# Autodesk Inventor assembly: コックピット_1
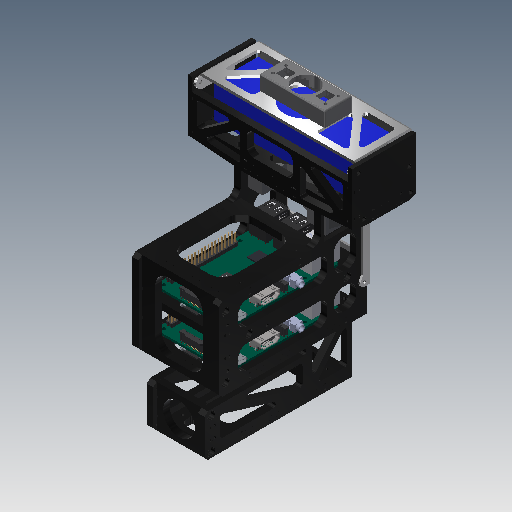
[picture p0: Inventor's stored thumbnail of the model, 512x512]
Saved by Autodesk Inventor 2017.3 (Build 213256000, 256)
## iProperties
Created: 2016-05-08
Part Number: コックピット_1
Document SubType Name: Assembly
Designer: hiroaki
Mass: 626.642 g
Surface Area: 2154.4 cm^2
Volume: 306.453 cm^3
Density: 2.04482 g/cm^3
Author: hiroaki
## Documents named in this file (19)
- C:\Users\haya\Desktop\GankenKun0_5\上半身\コックピット\コックピット_2\コックピット_2.iam
- C:\Users\haya\Desktop\GankenKun0_5\インポートされたコンポーネント\raspberrypi_b_+_(assembly)\raspberrypi_b_+_(assembly).iam
- C:\Users\haya\Desktop\GankenKun0_5\既製品\バッテリー(G6 HI-VOLTAGE 2400MAH 3S 80CMAX LIPO).ipt
- C:\Users\haya\Desktop\GankenKun0_5\既製品\sw.ipt
- C:\Users\haya\Desktop\GankenKun0_5\上半身\コックピット\コックピット_2\コックピット_サブフレーム_1_3.ipt
- C:\Users\haya\Desktop\GankenKun0_5\上半身\コックピット\コックピット_2\コックピット_サブフレーム_1_5.ipt
- C:\Users\haya\Desktop\GankenKun0_5\上半身\コックピット\コックピット_2\コックピット_サブフレーム_1_6.ipt
- C:\Users\haya\Desktop\GankenKun0_5\上半身\コックピット\コックピット_2\コックピット_サブフレーム_1_7.ipt
- C:\Users\haya\Desktop\GankenKun0_5\上半身\コックピット\コックピット_2\コックピット_2_メインフレーム_1.ipt
- C:\Users\haya\Desktop\GankenKun0_5\上半身\コックピット\コックピット_2\コックピット_2_メインフレーム_1_MIR.ipt
- C:\Users\haya\Desktop\GankenKun0_5\上半身\コックピット\コックピット_2\コックピット_2_サブフレーム_1.ipt
- C:\Users\haya\Desktop\GankenKun0_5\上半身\コックピット\コックピット_2\コックピット_2_サブフレーム_2.ipt
- C:\Users\haya\Desktop\GankenKun0_5\上半身\コックピット\コックピット_2\コックピット_2_サブフレーム_3.ipt
- C:\Users\haya\Desktop\GankenKun0_5\上半身\コックピット\コックピット_2\コックピット_2_サブフレーム_4.ipt
- C:\Users\haya\Desktop\GankenKun0_5\上半身\コックピット\コックピット_2\コックピット_2_メインフレーム_2.ipt
- C:\Users\haya\Desktop\GankenKun0_5\上半身\コックピット\コックピット_2\コックピット_2_サブフレーム_5.ipt
- C:\Users\haya\Desktop\GankenKun0_5\上半身\コックピット\コックピット_2\コックピット_2_サブフレーム_6.ipt
- C:\Users\haya\Desktop\GankenKun0_5\既製品\New_Accelite_Controller_Cover.ipt
- C:\Users\haya\Desktop\GankenKun0_5\上半身\コックピット\コックピット_2\コックピット_サブフレーム_1_8.ipt
## Components (22 placed, 18 different names)
1. raspberrypi_b_+_(assembly):1 [sub-assembly] — メイト:34, メイト:35, メイト:36, メイト:37, メイト:38, メイト:47, メイト:48
2. raspberrypi_b_+_(assembly):2 [sub-assembly] — メイト:39, メイト:40, メイト:41, メイト:42, フラッシュ:10
3. バッテリー(G6 HI-VOLTAGE 2400MAH 3S 80CMAX LIPO):1 — メイト:8, メイト:12, フラッシュ:1
4. sw:1 — フラッシュ:8, フラッシュ:9, メイト:20, メイト:21, メイト:22
5. sw:2 — フラッシュ:8, フラッシュ:9, メイト:23
6. コックピット_サブフレーム_1_3:1 — メイト:12, フラッシュ:1, 挿入:21, 挿入:22, メイト:14, メイト:15, メイト:17, メイト:19, 挿入:40, 挿入:41, 挿入:42, 挿入:43
7. コックピット_サブフレーム_1_5:1 — 挿入:21, 挿入:22, メイト:16, 挿入:24, 挿入:39
8. コックピット_サブフレーム_1_6:1 — メイト:14, メイト:15, メイト:16, メイト:18
9. コックピット_サブフレーム_1_5:2 — メイト:17, メイト:18, メイト:19, 挿入:23, 挿入:25
10. コックピット_サブフレーム_1_7:1 — 挿入:23, 挿入:24, 挿入:25, 挿入:39, メイト:49, メイト:50, メイト:51, メイト:52
11. コックピット_2_メインフレーム_1:1 — メイト:20, メイト:21, メイト:22, 挿入:40, 挿入:41, メイト:24, メイト:25, メイト:26, メイト:29, メイト:30, メイト:31, メイト:32, 挿入:44, 挿入:45, 挿入:48, 挿入:49, メイト:53, メイト:54
12. コックピット_2_メインフレーム_1_MIR:1 — 挿入:42, 挿入:43, メイト:23, メイト:27, メイト:28, メイト:33, 挿入:46, 挿入:47, 挿入:50, 挿入:51, 挿入:60, 挿入:61
13. コックピット_2_サブフレーム_1:1 — メイト:24, メイト:25, メイト:26, メイト:27
14. コックピット_2_サブフレーム_2:1 — メイト:28, メイト:29, メイト:30, メイト:31, メイト:32, メイト:33, メイト:34, メイト:35, メイト:36, メイト:37, メイト:38, 挿入:52, 挿入:53, 挿入:54, 挿入:55
15. コックピット_2_サブフレーム_3:1 — メイト:39, メイト:40, メイト:41, メイト:42, 挿入:44, 挿入:45, 挿入:46, 挿入:47
16. コックピット_2_サブフレーム_4:1 — 挿入:48, 挿入:49, 挿入:50, 挿入:51
17. コックピット_2_メインフレーム_2:1 — 挿入:54, 挿入:55, メイト:44, メイト:45, 挿入:56, 挿入:57
18. コックピット_2_メインフレーム_2:2 — 挿入:52, 挿入:53, メイト:43, メイト:46, 挿入:58, 挿入:59
19. コックピット_2_サブフレーム_5:1 — メイト:43, メイト:44, メイト:45, メイト:46
20. コックピット_2_サブフレーム_6:1 — 挿入:56, 挿入:57, 挿入:58, 挿入:59
21. New_Accelite_Controller_Cover:1 — メイト:49, メイト:50, メイト:51, メイト:52
22. コックピット_サブフレーム_1_8:1 — 挿入:60, 挿入:61, メイト:53, メイト:54
## Relationships (75: Mate 43, Insert 28, Flush 4)
- メイト:8 [Mate] (-52.5 mm): バッテリー(G6 HI-VOLTAGE 2400MAH 3S 80CMAX LIPO):1
- メイト:12 [Mate] (5 mm): バッテリー(G6 HI-VOLTAGE 2400MAH 3S 80CMAX LIPO):1 ↔ コックピット_サブフレーム_1_3:1
- フラッシュ:1 [Flush] (5 mm): バッテリー(G6 HI-VOLTAGE 2400MAH 3S 80CMAX LIPO):1 ↔ コックピット_サブフレーム_1_3:1
- 挿入:21 [Insert]: コックピット_サブフレーム_1_3:1 ↔ コックピット_サブフレーム_1_5:1
- 挿入:22 [Insert]: コックピット_サブフレーム_1_3:1 ↔ コックピット_サブフレーム_1_5:1
- メイト:14 [Mate] (0.05 mm): コックピット_サブフレーム_1_3:1 ↔ コックピット_サブフレーム_1_6:1
- メイト:15 [Mate]: コックピット_サブフレーム_1_3:1 ↔ コックピット_サブフレーム_1_6:1
- メイト:16 [Mate]: コックピット_サブフレーム_1_5:1 ↔ コックピット_サブフレーム_1_6:1
- メイト:17 [Mate]: コックピット_サブフレーム_1_3:1 ↔ コックピット_サブフレーム_1_5:2
- メイト:18 [Mate] (0.05 mm): コックピット_サブフレーム_1_6:1 ↔ コックピット_サブフレーム_1_5:2
- メイト:19 [Mate] (0.05 mm): コックピット_サブフレーム_1_3:1 ↔ コックピット_サブフレーム_1_5:2
- 挿入:23 [Insert]: コックピット_サブフレーム_1_5:2 ↔ コックピット_サブフレーム_1_7:1
- 挿入:24 [Insert]: コックピット_サブフレーム_1_5:1 ↔ コックピット_サブフレーム_1_7:1
- 挿入:25 [Insert]: コックピット_サブフレーム_1_5:2 ↔ コックピット_サブフレーム_1_7:1
- フラッシュ:8 [Flush]: sw:1 ↔ sw:2
- フラッシュ:9 [Flush]: sw:1 ↔ sw:2
- 挿入:39 [Insert]: コックピット_サブフレーム_1_5:1 ↔ コックピット_サブフレーム_1_7:1
- メイト:20 [Mate]: sw:1 ↔ コックピット_2_メインフレーム_1:1
- メイト:21 [Mate] (0.55 mm): sw:1 ↔ コックピット_2_メインフレーム_1:1
- メイト:22 [Mate] (0.3 mm): sw:1 ↔ コックピット_2_メインフレーム_1:1
- 挿入:40 [Insert]: コックピット_サブフレーム_1_3:1 ↔ コックピット_2_メインフレーム_1:1
- 挿入:41 [Insert]: コックピット_サブフレーム_1_3:1 ↔ コックピット_2_メインフレーム_1:1
- 挿入:42 [Insert]: コックピット_サブフレーム_1_3:1 ↔ コックピット_2_メインフレーム_1_MIR:1
- 挿入:43 [Insert]: コックピット_サブフレーム_1_3:1 ↔ コックピット_2_メインフレーム_1_MIR:1
- メイト:23 [Mate]: sw:2 ↔ コックピット_2_メインフレーム_1_MIR:1
- メイト:24 [Mate] (0.05 mm): コックピット_2_メインフレーム_1:1 ↔ コックピット_2_サブフレーム_1:1
- メイト:25 [Mate] (0.05 mm): コックピット_2_メインフレーム_1:1 ↔ コックピット_2_サブフレーム_1:1
- メイト:26 [Mate]: コックピット_2_メインフレーム_1:1 ↔ コックピット_2_サブフレーム_1:1
- メイト:27 [Mate]: コックピット_2_メインフレーム_1_MIR:1 ↔ コックピット_2_サブフレーム_1:1
- メイト:28 [Mate]: コックピット_2_メインフレーム_1_MIR:1 ↔ コックピット_2_サブフレーム_2:1
- メイト:29 [Mate]: コックピット_2_メインフレーム_1:1 ↔ コックピット_2_サブフレーム_2:1
- メイト:30 [Mate] (0.05 mm): コックピット_2_メインフレーム_1:1 ↔ コックピット_2_サブフレーム_2:1
- メイト:31 [Mate] (0.05 mm): コックピット_2_メインフレーム_1:1 ↔ コックピット_2_サブフレーム_2:1
- メイト:32 [Mate] (0.05 mm): コックピット_2_メインフレーム_1:1 ↔ コックピット_2_サブフレーム_2:1
- メイト:33 [Mate] (0.05 mm): コックピット_2_メインフレーム_1_MIR:1 ↔ コックピット_2_サブフレーム_2:1
- メイト:34 [Mate]: raspberrypi_b_+_(assembly):1 ↔ コックピット_2_サブフレーム_2:1
- メイト:35 [Mate]: raspberrypi_b_+_(assembly):1 ↔ コックピット_2_サブフレーム_2:1
- メイト:36 [Mate]: raspberrypi_b_+_(assembly):1 ↔ コックピット_2_サブフレーム_2:1
- メイト:37 [Mate]: raspberrypi_b_+_(assembly):1 ↔ コックピット_2_サブフレーム_2:1
- メイト:38 [Mate] (3 mm): raspberrypi_b_+_(assembly):1 ↔ コックピット_2_サブフレーム_2:1
- メイト:39 [Mate]: raspberrypi_b_+_(assembly):2 ↔ コックピット_2_サブフレーム_3:1
- メイト:40 [Mate] (3 mm): raspberrypi_b_+_(assembly):2 ↔ コックピット_2_サブフレーム_3:1
- メイト:41 [Mate]: raspberrypi_b_+_(assembly):2 ↔ コックピット_2_サブフレーム_3:1
- メイト:42 [Mate]: raspberrypi_b_+_(assembly):2 ↔ コックピット_2_サブフレーム_3:1
- 挿入:44 [Insert]: コックピット_2_メインフレーム_1:1 ↔ コックピット_2_サブフレーム_3:1
- 挿入:45 [Insert]: コックピット_2_メインフレーム_1:1 ↔ コックピット_2_サブフレーム_3:1
- 挿入:46 [Insert]: コックピット_2_メインフレーム_1_MIR:1 ↔ コックピット_2_サブフレーム_3:1
- 挿入:47 [Insert]: コックピット_2_メインフレーム_1_MIR:1 ↔ コックピット_2_サブフレーム_3:1
- 挿入:48 [Insert]: コックピット_2_メインフレーム_1:1 ↔ コックピット_2_サブフレーム_4:1
- 挿入:49 [Insert]: コックピット_2_メインフレーム_1:1 ↔ コックピット_2_サブフレーム_4:1
- 挿入:50 [Insert]: コックピット_2_メインフレーム_1_MIR:1 ↔ コックピット_2_サブフレーム_4:1
- 挿入:51 [Insert]: コックピット_2_メインフレーム_1_MIR:1 ↔ コックピット_2_サブフレーム_4:1
- 挿入:52 [Insert]: コックピット_2_サブフレーム_2:1 ↔ コックピット_2_メインフレーム_2:2
- 挿入:53 [Insert]: コックピット_2_サブフレーム_2:1 ↔ コックピット_2_メインフレーム_2:2
- 挿入:54 [Insert]: コックピット_2_サブフレーム_2:1 ↔ コックピット_2_メインフレーム_2:1
- 挿入:55 [Insert]: コックピット_2_サブフレーム_2:1 ↔ コックピット_2_メインフレーム_2:1
- メイト:43 [Mate] (0.05 mm): コックピット_2_メインフレーム_2:2 ↔ コックピット_2_サブフレーム_5:1
- メイト:44 [Mate] (0.05 mm): コックピット_2_メインフレーム_2:1 ↔ コックピット_2_サブフレーム_5:1
- メイト:45 [Mate]: コックピット_2_メインフレーム_2:1 ↔ コックピット_2_サブフレーム_5:1
- メイト:46 [Mate]: コックピット_2_メインフレーム_2:2 ↔ コックピット_2_サブフレーム_5:1
- メイト:47 [Mate] (-28 mm): raspberrypi_b_+_(assembly):1
- フラッシュ:10 [Flush] (42.5 mm): raspberrypi_b_+_(assembly):2
- メイト:48 [Mate]: raspberrypi_b_+_(assembly):1
- 挿入:56 [Insert]: コックピット_2_メインフレーム_2:1 ↔ コックピット_2_サブフレーム_6:1
- 挿入:57 [Insert]: コックピット_2_メインフレーム_2:1 ↔ コックピット_2_サブフレーム_6:1
- 挿入:58 [Insert]: コックピット_2_メインフレーム_2:2 ↔ コックピット_2_サブフレーム_6:1
- 挿入:59 [Insert]: コックピット_2_メインフレーム_2:2 ↔ コックピット_2_サブフレーム_6:1
- メイト:49 [Mate]: コックピット_サブフレーム_1_7:1 ↔ New_Accelite_Controller_Cover:1
- メイト:50 [Mate]: コックピット_サブフレーム_1_7:1 ↔ New_Accelite_Controller_Cover:1
- メイト:51 [Mate]: コックピット_サブフレーム_1_7:1 ↔ New_Accelite_Controller_Cover:1
- メイト:52 [Mate]: コックピット_サブフレーム_1_7:1 ↔ New_Accelite_Controller_Cover:1
- 挿入:60 [Insert]: コックピット_2_メインフレーム_1_MIR:1 ↔ コックピット_サブフレーム_1_8:1
- 挿入:61 [Insert]: コックピット_2_メインフレーム_1_MIR:1 ↔ コックピット_サブフレーム_1_8:1
- メイト:53 [Mate]: コックピット_2_メインフレーム_1:1 ↔ コックピット_サブフレーム_1_8:1
- メイト:54 [Mate]: コックピット_2_メインフレーム_1:1 ↔ コックピット_サブフレーム_1_8:1
